# Autodesk Inventor assembly: Standard Wheel Assembly V3
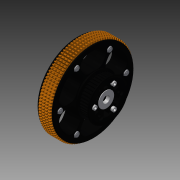
[picture p0: Inventor's stored thumbnail of the model, 180x180]
Saved by Autodesk Inventor 2014 SP1 (Build 180222100, 222)
## iProperties
Created: 2013-01-17
Part Number: Standard Wheel Assembly V3
Document SubType Name: Assembly
Designer: Moses
Mass: 509.063 g
Surface Area: 1705.29 cm^2
Volume: 364.57 cm^3
Density: 1.39634 g/cm^3
Author: Moses
## Documents named in this file (6)
- C:\Users\Moses\Documents\Inventor\Sally Rebuild\Rebuild Sally\Standard Wheel Assembly V3.iam
- C:\Users\Moses\Documents\Inventor\Sally Rebuild\Rebuild Sally\DBK_42ToothPulley V2.iam
- C:\Users\Moses\Documents\Inventor\Sally Rebuild\Rebuild Sally\r8 bearing.ipt
- C:\Users\Moses\Documents\Inventor\Sally Rebuild\Rebuild Sally\91251A255.ipt
- C:\Users\Moses\Documents\Inventor\Sally Rebuild\Rebuild Sally\91831A011.ipt
- C:\Users\Moses\Documents\Inventor\Sally Rebuild\Rebuild Sally\6Plaction-asm V2.iam
## Components (10 placed, 5 different names)
1. 6Plaction-asm V2:1 [sub-assembly] — Mate:2, Mate:3, Insert:8, Tangent:1, Insert:12, Insert:13, Insert:14, Angle:1, Angle:2, Angle:3
2. DBK_42ToothPulley V2:2 [sub-assembly] — Mate:2, Mate:3, Insert:7, Insert:9, Insert:10, Insert:11, Tangent:1
3. r8 bearing:1 — Insert:7
4. r8 bearing:2 — Insert:8
5. 91251A255:1 — Insert:9
6. 91251A255:2 — Insert:10
7. 91251A255:3 — Insert:11
8. 91831A011:1 — Insert:12, Angle:1
9. 91831A011:2 — Insert:13, Angle:3
10. 91831A011:3 — Insert:14, Angle:2
## Relationships (14: Insert 8, Angle 3, Mate 2, Tangent 1)
- Mate:2: 6Plaction-asm V2:1 ↔ DBK_42ToothPulley V2:2
- Mate:3: 6Plaction-asm V2:1 ↔ DBK_42ToothPulley V2:2
- Insert:7: DBK_42ToothPulley V2:2 ↔ r8 bearing:1
- Insert:8: 6Plaction-asm V2:1 ↔ r8 bearing:2
- Insert:9: DBK_42ToothPulley V2:2 ↔ 91251A255:1
- Insert:10: DBK_42ToothPulley V2:2 ↔ 91251A255:2
- Insert:11: DBK_42ToothPulley V2:2 ↔ 91251A255:3
- Tangent:1: 6Plaction-asm V2:1 ↔ DBK_42ToothPulley V2:2
- Insert:12: 6Plaction-asm V2:1 ↔ 91831A011:1
- Insert:13: 6Plaction-asm V2:1 ↔ 91831A011:2
- Insert:14: 6Plaction-asm V2:1 ↔ 91831A011:3
- Angle:1 (90 deg): 6Plaction-asm V2:1 ↔ 91831A011:1
- Angle:2 (90 deg): 6Plaction-asm V2:1 ↔ 91831A011:3
- Angle:3 (90 deg): 6Plaction-asm V2:1 ↔ 91831A011:2
